# Autodesk Inventor assembly: ASY MSC 122  base frame
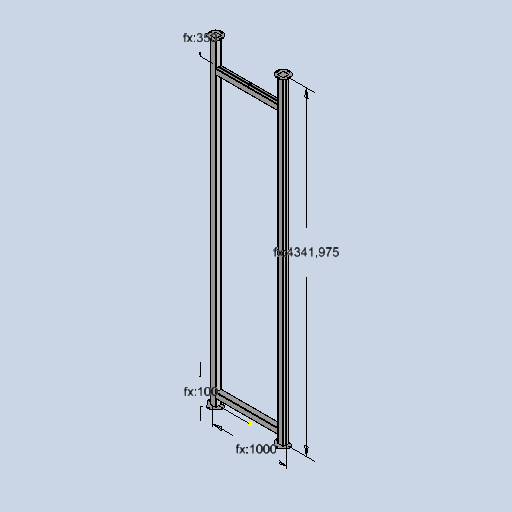
[picture p0: Inventor's stored thumbnail of the model, 512x512]
Saved by Autodesk Inventor 2025 (Build 290162010, 162A)
## iProperties
_SolveAssemblyDoc: Frame Generator Solve Assembly
_Version: 25.0.0
Created: 2024-06-30
Part Number: ASY MSC 122  base frame
Document SubType Name: Assembly
Designer: pokla
Stock Number: ASY МОО 122 базовая рама
Author: pokla
## Documents named in this file (5)
- C:\Users\pokla\Documents\Inventor\Отстойник осветлитель\Manturovo_Se-clar-Gleb\ASY MSC 122  base frame.iam
- C:\Users\pokla\Documents\Inventor\Отстойник осветлитель\Manturovo_Se-clar-Gleb\ASY MSC 122  base frame.ipt
- C:\Users\pokla\Documents\Inventor\Отстойник осветлитель\Manturovo_Se-clar-Gleb\ASY MSC 122  base frame\Frame\Frame 1719749399381.iam
- C:\Users\pokla\Documents\Inventor\Отстойник осветлитель\Manturovo_Se-clar-Gleb\MSC 127 flange frame heel.ipt
- C:\Users\pokla\Documents\Inventor\Отстойник осветлитель\Manturovo_Se-clar-Gleb\MSC 126 flange frame.ipt
## Components (6 placed, 4 different names)
1. ASY MSC 122  base frame:1
2. Frame 1719749399381:1 [sub-assembly] — Rigid:1, Rigid:2, Rigid:3, Rigid:4
3. MSC 127 flange frame heel:1 — Rigid:1
4. MSC 127 flange frame heel:2 — Rigid:2
5. MSC 126 flange frame:1 — Rigid:3
6. MSC 126 flange frame:2 — Rigid:4
## Relationships (4: WeldJoint 4)
- Rigid:1 [WeldJoint]: Frame 1719749399381:1 ↔ MSC 127 flange frame heel:1
- Rigid:2 [WeldJoint]: Frame 1719749399381:1 ↔ MSC 127 flange frame heel:2
- Rigid:3 [WeldJoint]: Frame 1719749399381:1 ↔ MSC 126 flange frame:1
- Rigid:4 [WeldJoint]: Frame 1719749399381:1 ↔ MSC 126 flange frame:2
